# Autodesk Inventor assembly: Sterics-Assembly
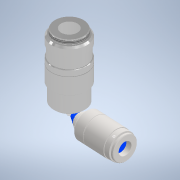
[picture p0: Inventor's stored thumbnail of the model, 180x180]
Saved by Autodesk Inventor 2022 (Build 260153000, 153)
## iProperties
Created: 2020-10-21
Part Number: Sterics-Assembly
Document SubType Name: Assembly
Designer: MicroscopyInnovation
Author: MicroscopyInnovation
## Documents named in this file (4)
- C:\Users\Spectral\Documents\GitHub\CAD\Manuscripts\Lattice_Sample_Handling\Sterics-Assembly.iam
- C:\Users\Spectral\Documents\GitHub\CAD\components\SpecialOptics\54-10-7.ipt
- C:\Users\Spectral\Documents\GitHub\CAD\components\Nikon\N25XW-Apo-LWD-NA1pt1.ipt
- C:\Users\Spectral\Documents\GitHub\CAD\components\HarvardApparatus\64-0700.ipt
## Components (3 placed, 3 different names)
1. 54-10-7:1 — Mate:1, Angle:2, Mate:2, Mate:4, Angle:3
2. N25XW-Apo-LWD-NA1pt1:1 — Mate:1, Angle:2, Mate:2, Mate:3
3. 64-0700:1 — Mate:3, Mate:4, Angle:3
## Relationships (6: Mate 4, Angle 2)
- Mate:1 (2 mm): 54-10-7:1 ↔ N25XW-Apo-LWD-NA1pt1:1
- Angle:2 (90 deg): 54-10-7:1 ↔ N25XW-Apo-LWD-NA1pt1:1
- Mate:2 (3.74 mm): 54-10-7:1 ↔ N25XW-Apo-LWD-NA1pt1:1
- Mate:3: N25XW-Apo-LWD-NA1pt1:1 ↔ 64-0700:1
- Mate:4: 54-10-7:1 ↔ 64-0700:1
- Angle:3 (58.2 deg): 54-10-7:1 ↔ 64-0700:1
